# Autodesk Inventor assembly: Full Door
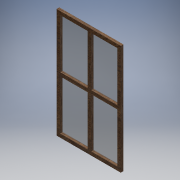
[picture p0: Inventor's stored thumbnail of the model, 180x180]
Saved by Autodesk Inventor 2017 (Build 210142000, 142)
## iProperties
Created: 2016-09-13
Part Number: Full Door
Document SubType Name: Assembly
Designer: s.ethan.wierenga
Author: s.ethan.wierenga
## Documents named in this file (3)
- E:\Github\home\ahri\.freepantry\.files\Full Door.iam
- E:\Github\home\ahri\.freepantry\.files\Door.ipt
- E:\Github\home\ahri\.freepantry\.files\Glass Sheet.ipt
## Components (2 placed, 2 different names)
1. Door:1 — Flush:1, Flush:2, Flush:3
2. Glass Sheet:1 — Flush:1, Flush:2, Flush:3
## Relationships (3: Flush 3)
- Flush:1 (19.05 mm): Door:1 ↔ Glass Sheet:1
- Flush:2 (19.05 mm): Door:1 ↔ Glass Sheet:1
- Flush:3: Door:1 ↔ Glass Sheet:1
